# Autodesk Inventor assembly: 2016-01-25-RhinoRobot
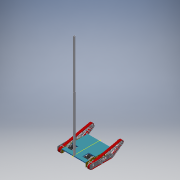
[picture p0: Inventor's stored thumbnail of the model, 180x180]
Saved by Autodesk Inventor 2016 SP1 (Build 200210100, 210)
## iProperties
Created: 2016-01-23
Part Number: 2016-01-25-RhinoRobot
Document SubType Name: Assembly
Designer: steele
Mass: 10784.8 g
Surface Area: 26494.6 cm^2
Volume: 9600.19 cm^3
Density: 1.12339 g/cm^3
Author: steele
## Documents named in this file (6)
- C:\snobotics\CAD-Development\robSteele\SnoBotics2016\2016-01-25-RhinoRobot\2016-01-25-RhinoRobot.iam
- C:\snobotics\CAD-Development\robSteele\SnoBotics2016\RhinoTrackDriveModule\am-3322+RhinoTrackDriveModule.iam
- C:\snobotics\CAD-Development\robSteele\SnoBotics2016\RhinoBottomFloorOptions\RhinoBottomFloorPlate03.ipt
- C:\snobotics\CAD-Development\robSteele\SnoBotics2016\RhinoTrackDriveModule\am-3322+RhinoTrackDriveModule_MIR6.iam
- C:\snobotics\CAD-Development\robSteele\SnoBotics2016\TelescopeArm\1_250_inchSquareTube.ipt
- C:\snobotics\CAD-Development\robSteele\SnoBotics2016\TelescopeArm\1_000_inchSquareTube.ipt
## Components (5 placed, 5 different names)
1. RhinoBottomFloorPlate03:1 — Mate:1, Flush:2, Flush:3, Mate:2, Mate:3, Mate:4
2. am-3322+RhinoTrackDriveModule:1 [sub-assembly] — Mate:1, Flush:2, Flush:3
3. am-3322+RhinoTrackDriveModule_MIR6:1 [sub-assembly]
4. 1_250_inchSquareTube:1 — Mate:2, Mate:3, Mate:4, Mate:5, Mate:6, Mate:7
5. 1_000_inchSquareTube:1 — Mate:5, Mate:6, Mate:7
## Relationships (9: Mate 7, Flush 2)
- Mate:1 (3.175 mm): RhinoBottomFloorPlate03:1 ↔ am-3322+RhinoTrackDriveModule:1
- Flush:2: RhinoBottomFloorPlate03:1 ↔ am-3322+RhinoTrackDriveModule:1
- Flush:3: RhinoBottomFloorPlate03:1 ↔ am-3322+RhinoTrackDriveModule:1
- Mate:2: RhinoBottomFloorPlate03:1 ↔ 1_250_inchSquareTube:1
- Mate:3: RhinoBottomFloorPlate03:1 ↔ 1_250_inchSquareTube:1
- Mate:4: RhinoBottomFloorPlate03:1 ↔ 1_250_inchSquareTube:1
- Mate:5 (-127 mm): 1_250_inchSquareTube:1 ↔ 1_000_inchSquareTube:1
- Mate:6: 1_250_inchSquareTube:1 ↔ 1_000_inchSquareTube:1
- Mate:7: 1_250_inchSquareTube:1 ↔ 1_000_inchSquareTube:1
## Named parameters: robotWidth = 660.4 mm, halfRobotWidth = 330.2 mm, maxPerimeter = 3048 mm, maxLength = 863.6 mm, widthOfTrack = 95.25 mm, boardWidth = 469.9 mm
